# Autodesk Inventor assembly: Analiza naprężeń
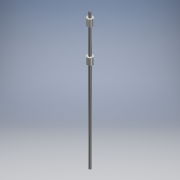
[picture p0: Inventor's stored thumbnail of the model, 180x180]
Saved by Autodesk Inventor 2019.4 (Build 234330000, 330)
## iProperties
Created: 2020-08-31
Part Number: Analiza naprężeń
Material: Ogólny
Document SubType Name: Assembly
Designer: barto
Author: barto
## Documents named in this file (10)
- F:\GitHub\MUMv2\Equatorial-Mount-MUM\Mechanika\Moduł obrotu DEK Bartek\odBartka\Analiza naprężeń.iam
- F:\GitHub\MUMv2\Equatorial-Mount-MUM\Mechanika\Moduł obrotu RET Estera\projejt\projejt\NoweZlozenie\walekREK.ipt
- C:\Users\barto\OneDrive\Pulpit\Część2.ipt
- F:\GitHub\MUMv2\Equatorial-Mount-MUM\Mechanika\Moduł obrotu DEK Bartek\odBartka\Analiza naprężeń\AIP\FEA\dcld90ykg.fins
- F:\GitHub\MUMv2\Equatorial-Mount-MUM\Mechanika\Moduł obrotu DEK Bartek\odBartka\Analiza naprężeń\AIP\FEA\dcld90ykg.fsat
- F:\GitHub\MUMv2\Equatorial-Mount-MUM\Mechanika\Moduł obrotu DEK Bartek\odBartka\Analiza naprężeń\AIP\FEA\dcld90ykg.ftes
- F:\GitHub\MUMv2\Equatorial-Mount-MUM\Mechanika\Moduł obrotu DEK Bartek\odBartka\Analiza naprężeń\AIP\FEA\dcld90ykg.fwiz
- F:\GitHub\MUMv2\Equatorial-Mount-MUM\Mechanika\Moduł obrotu DEK Bartek\odBartka\Analiza naprężeń\AIP\FEA\dcld90yn4.fmsh
- F:\GitHub\MUMv2\Equatorial-Mount-MUM\Mechanika\Moduł obrotu DEK Bartek\odBartka\Analiza naprężeń\AIP\FEA\dcld90yn5.fres
- F:\GitHub\MUMv2\Equatorial-Mount-MUM\Mechanika\Moduł obrotu DEK Bartek\odBartka\Analiza naprężeń\AIP\FEA\dcmutmkhs.fres
## Components (3 placed, 2 different names)
1. walekREK:1 — Zestawiające:1, Zestawiające:2, Równoległe:1, Równoległe:2
2. Część2:1 — Zestawiające:1, Równoległe:2
3. Część2:2 — Zestawiające:2, Równoległe:1
## Relationships (4: Mate 2, Flush 2)
- Zestawiające:1 [Mate]: walekREK:1 ↔ Część2:1
- Zestawiające:2 [Mate]: walekREK:1 ↔ Część2:2
- Równoległe:1 [Flush]: walekREK:1 ↔ Część2:2
- Równoległe:2 [Flush]: walekREK:1 ↔ Część2:1
## Named parameters: sa_0 = 10000, sa_1 = 0, sa_2 = 0, sa_3 = 10000, sa_4 = 0, sa_5 = 0
note: some values were not read from the file. Shown as the stored number, unit unknown: "sa_0", "sa_1", "sa_2", "sa_3", "sa_4", "sa_5".
